# Autodesk Inventor assembly: Assembly1
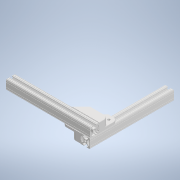
[picture p0: Inventor's stored thumbnail of the model, 180x180]
Saved by Autodesk Inventor 2020 (Build 240168000, 168)
## iProperties
Created: 2020-01-08
Part Number: Assembly1
Document SubType Name: Assembly
Designer: srini
Author: srini
## Documents named in this file (3)
- C:\Users\srini\Documents\FRC\2020\Assembly1.iam
- C:\Users\srini\Documents\FRC\2020\1003-9-CL.ipt
- C:\Users\srini\Documents\FRC\2020\90DegJoiner.ipt
## Components (3 placed, 2 different names)
1. 1003-9-CL:1 — Flush:2, Flush:4, Flush:5, Mate:1
2. 1003-9-CL:2 — Flush:2, Flush:3, Flush:5, Mate:1
3. 90DegJoiner:1 — Flush:3, Flush:4
## Relationships (5: Flush 4, Mate 1)
- Flush:2: 1003-9-CL:1 ↔ 1003-9-CL:2
- Flush:3: 1003-9-CL:2 ↔ 90DegJoiner:1
- Flush:4: 1003-9-CL:1 ↔ 90DegJoiner:1
- Flush:5: 1003-9-CL:1 ↔ 1003-9-CL:2
- Mate:1: 1003-9-CL:1 ↔ 1003-9-CL:2
